# Autodesk Inventor assembly: MecanismoBloq2
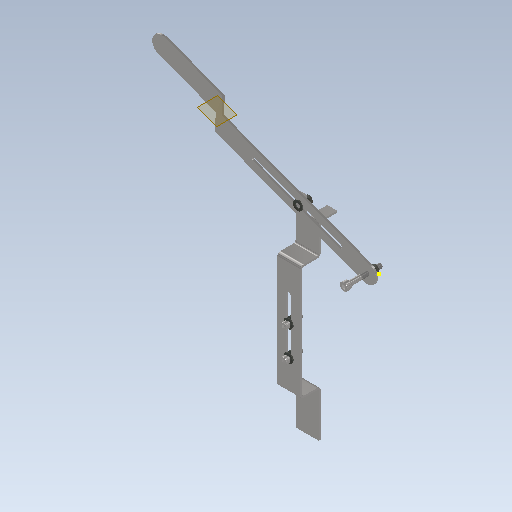
[picture p0: Inventor's stored thumbnail of the model, 512x512]
Saved by Autodesk Inventor 2021 (Build 250183000, 183)
## iProperties
Created: 2021-06-10
Part Number: MecanismoBloq2
Document SubType Name: Assembly
Designer: GABRIEL LOL
Author: GABRIEL LOL
## Documents named in this file (8)
- E:\Documentos\Documentos\Michael_Rodriguez\Universidad_Nacional\Doceaba matricula\PAI\Proyecto PAI\Proyecto_PAI_2021\01 CAD\mecanismobloq2\MecanismoBloq2.iam
- E:\Documentos\Documentos\Michael_Rodriguez\Universidad_Nacional\Doceaba matricula\PAI\Proyecto PAI\Proyecto_PAI_2021\01 CAD\mecanismobloq2\PalancaAccionMecBloq2.ipt
- E:\Documentos\Documentos\Michael_Rodriguez\Universidad_Nacional\Doceaba matricula\PAI\Proyecto PAI\Proyecto_PAI_2021\01 CAD\mecanismobloq2\PistaMecBloq2.ipt
- C:\Users\GABRIEL LOL\Documents\Inventor\Content Center Files\R2021\en-US\SS-ISO 4762\ISO 4762 - M5 x 16SS-ISO.ipt
- E:\Documentos\Documentos\Michael_Rodriguez\Universidad_Nacional\Doceaba matricula\PAI\Proyecto PAI\Proyecto_PAI_2021\01 CAD\mecanismobloq2\ISO 8738 - 5.ipt
- E:\Documentos\Documentos\Michael_Rodriguez\Universidad_Nacional\Doceaba matricula\PAI\Proyecto PAI\Proyecto_PAI_2021\01 CAD\mecanismobloq2\ISO 7041 - M5SS-ISO.ipt
- E:\Documentos\Documentos\Michael_Rodriguez\Universidad_Nacional\Doceaba matricula\PAI\Proyecto PAI\Proyecto_PAI_2021\01 CAD\mecanismobloq2\ISO 4762 - M4 x 16SS-ISO.ipt
- E:\Documentos\Documentos\Michael_Rodriguez\Universidad_Nacional\Doceaba matricula\PAI\Proyecto PAI\Proyecto_PAI_2021\01 CAD\mecanismobloq2\ISO 4762 - M5 x 35SS-ISO.ipt
## Components (15 placed, 7 different names)
1. PalancaAccionMecBloq2:1 — Tangent:1, Mate:5, Mate:6, Mate:23, Mate:24, Mate:26
2. PistaMecBloq2:1 — Mate:2, Mate:6, Mate:8, Angle:1, Tangent:2, Tangent:3, Mate:11, Tangent:4, Mate:14, Mate:17, Mate:18
3. SS ISO 4762 M5 x 35:1 — Mate:23, Mate:24, Mate:25
4. SS ISO 4762 M4 x 16:1 — Tangent:2, Mate:9, Mate:10, Mate:15, Mate:19
5. SS ISO 4762 M4 x 16:2 — Tangent:3, Mate:12, Mate:13, Tangent:4, Mate:16, Mate:20
6. SS ISO 4762 M5 x 16:1 — Tangent:1, Mate:2, Mate:3, Mate:4, Mate:7
7. ISO 8738 5:1 — Mate:3, Mate:4, Mate:5
8. SS ISO 7041 M5:1 — Mate:7, Mate:8
9. ISO 8738 5:2 — Mate:9, Mate:10, Mate:11
10. ISO 8738 5:3 — Mate:12, Mate:13, Mate:14
11. ISO 8738 5:4 — Mate:15, Mate:17, Mate:22
12. ISO 8738 5:5 — Mate:16, Mate:18, Mate:21
13. SS ISO 7041 M5:2 — Mate:19, Mate:22
14. SS ISO 7041 M5:3 — Mate:20, Mate:21
15. SS ISO 7041 M5:4 — Mate:25, Mate:26
## Relationships (30: Mate 25, Tangent 4, Angle 1)
- Tangent:1: PalancaAccionMecBloq2:1 ↔ SS ISO 4762 M5 x 16:1
- Mate:2: PistaMecBloq2:1 ↔ SS ISO 4762 M5 x 16:1
- Mate:3: SS ISO 4762 M5 x 16:1 ↔ ISO 8738 5:1
- Mate:4: SS ISO 4762 M5 x 16:1 ↔ ISO 8738 5:1
- Mate:5: PalancaAccionMecBloq2:1 ↔ ISO 8738 5:1
- Mate:6: PalancaAccionMecBloq2:1 ↔ PistaMecBloq2:1
- Mate:7: SS ISO 4762 M5 x 16:1 ↔ SS ISO 7041 M5:1
- Mate:8: PistaMecBloq2:1 ↔ SS ISO 7041 M5:1
- Angle:1 (180 deg): PistaMecBloq2:1
- Tangent:2: PistaMecBloq2:1 ↔ SS ISO 4762 M4 x 16:1
- Tangent:3: PistaMecBloq2:1 ↔ SS ISO 4762 M4 x 16:2
- Mate:9: SS ISO 4762 M4 x 16:1 ↔ ISO 8738 5:2
- Mate:10 (1.21 mm): SS ISO 4762 M4 x 16:1 ↔ ISO 8738 5:2
- Mate:11: PistaMecBloq2:1 ↔ ISO 8738 5:2
- Mate:12: SS ISO 4762 M4 x 16:2 ↔ ISO 8738 5:3
- Mate:13 (1.21 mm): SS ISO 4762 M4 x 16:2 ↔ ISO 8738 5:3
- Tangent:4: PistaMecBloq2:1 ↔ SS ISO 4762 M4 x 16:2
- Mate:14: PistaMecBloq2:1 ↔ ISO 8738 5:3
- Mate:15: SS ISO 4762 M4 x 16:1 ↔ ISO 8738 5:4
- Mate:16: SS ISO 4762 M4 x 16:2 ↔ ISO 8738 5:5
- Mate:17: PistaMecBloq2:1 ↔ ISO 8738 5:4
- Mate:18: PistaMecBloq2:1 ↔ ISO 8738 5:5
- Mate:19: SS ISO 4762 M4 x 16:1 ↔ SS ISO 7041 M5:2
- Mate:20: SS ISO 4762 M4 x 16:2 ↔ SS ISO 7041 M5:3
- Mate:21: ISO 8738 5:5 ↔ SS ISO 7041 M5:3
- Mate:22: ISO 8738 5:4 ↔ SS ISO 7041 M5:2
- Mate:23: PalancaAccionMecBloq2:1 ↔ SS ISO 4762 M5 x 35:1
- Mate:24 (20.1 mm): PalancaAccionMecBloq2:1 ↔ SS ISO 4762 M5 x 35:1
- Mate:25: SS ISO 4762 M5 x 35:1 ↔ SS ISO 7041 M5:4
- Mate:26: PalancaAccionMecBloq2:1 ↔ SS ISO 7041 M5:4
